# Autodesk Inventor assembly: ROBOT_1_4
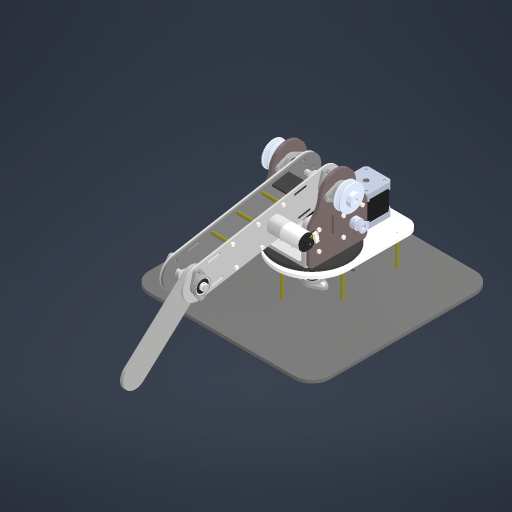
[picture p0: Inventor's stored thumbnail of the model, 512x512]
Saved by Autodesk Inventor 2023 (Build 270158000, 158)
## iProperties
Created: 2023-09-06
Part Number: ROBOT_1_4
Document SubType Name: Assembly
Designer: philo
Sending System: Autodesk Inventor 2023
Preprocessor: ST-DEVELOPER v19
Title: C:\Users\philo\OneDrive\Desktop\HK1-2024\TT ROBOT\3DVer2\ROBOT_1_2.stp
Author: philo
## Documents named in this file (28)
- C:\Users\philo\OneDrive\Desktop\HK1-2024\TT ROBOT\02_3D_design\ROBOT_1_4.iam
- C:\Users\philo\OneDrive\Desktop\HK1-2024\TT ROBOT\02_3D_design\DeRobot.ipt
- C:\Users\philo\OneDrive\Desktop\HK1-2024\TT ROBOT\02_3D_design\Detron.ipt
- C:\Users\philo\OneDrive\Desktop\HK1-2024\TT ROBOT\02_3D_design\goidoObi.ipt
- C:\Users\philo\OneDrive\Desktop\HK1-2024\TT ROBOT\02_3D_design\truday.ipt
- C:\Users\philo\OneDrive\Desktop\HK1-2024\TT ROBOT\02_3D_design\gt2_60teeth.iam
- C:\Users\philo\OneDrive\Desktop\HK1-2024\TT ROBOT\02_3D_design\STEP MOTOR NEMA 17.ipt
- C:\Users\philo\OneDrive\Desktop\HK1-2024\TT ROBOT\02_3D_design\GT2 Pulley 20 Tooth (ID6mm).ipt
- C:\Users\philo\OneDrive\Desktop\HK1-2024\TT ROBOT\02_3D_design\M3 x 5mm.ipt
- C:\Users\philo\OneDrive\Desktop\HK1-2024\TT ROBOT\02_3D_design\Diaquay.ipt
- C:\Users\philo\OneDrive\Desktop\HK1-2024\TT ROBOT\02_3D_design\Tb6600.ipt
- C:\Users\philo\OneDrive\Desktop\HK1-2024\TT ROBOT\02_3D_design\ESP-WROOM32.iam
- C:\Users\philo\OneDrive\Desktop\HK1-2024\TT ROBOT\02_3D_design\codinhtruc.ipt
- C:\Users\philo\OneDrive\Desktop\HK1-2024\TT ROBOT\02_3D_design\daydai.ipt
- C:\Users\philo\OneDrive\Desktop\HK1-2024\TT ROBOT\02_3D_design\gt2smooth.ipt
- C:\Users\philo\OneDrive\Desktop\HK1-2024\TT ROBOT\02_3D_design\trudong5mm.ipt
- C:\Users\philo\OneDrive\Desktop\HK1-2024\TT ROBOT\02_3D_design\trucdogt2.ipt
- C:\Users\philo\OneDrive\Desktop\HK1-2024\TT ROBOT\02_3D_design\HALL.ipt
- C:\Users\philo\OneDrive\Desktop\HK1-2024\TT ROBOT\02_3D_design\namcham.ipt
- C:\Users\philo\OneDrive\Desktop\HK1-2024\TT ROBOT\02_3D_design\Tamop1.ipt
- C:\Users\philo\OneDrive\Desktop\HK1-2024\TT ROBOT\02_3D_design\60pitch pulley GT2 6mm ASSEMBLY.iam
- C:\Users\philo\OneDrive\Desktop\HK1-2024\TT ROBOT\02_3D_design\truc8mm.ipt
- C:\Users\philo\OneDrive\Desktop\HK1-2024\TT ROBOT\02_3D_design\giulink2.ipt
- C:\Users\philo\OneDrive\Desktop\HK1-2024\TT ROBOT\02_3D_design\Link2Base.ipt
- C:\Users\philo\OneDrive\Desktop\HK1-2024\TT ROBOT\02_3D_design\thanhnang.ipt
- C:\Users\philo\OneDrive\Desktop\HK1-2024\TT ROBOT\02_3D_design\trudong3mm.ipt
- C:\Users\philo\OneDrive\Desktop\HK1-2024\TT ROBOT\02_3D_design\Link3base.ipt
- C:\Users\philo\OneDrive\Desktop\HK1-2024\TT ROBOT\02_3D_design\Dongco.iam
## Components (85 placed, 27 different names)
1. Link3base:1 — Mate:171, Flush:17
2. Dongco:1 [sub-assembly] — Mate:172, Angle:18
3. DeRobot:1 — Mate:81, Mate:82, Mate:83, Mate:84, Mate:85, Mate:86, Mate:87, Mate:90, Mate:91, Mate:92, Mate:95, ROBOTQUAY, Flush:16
4. Detron:1 — Mate:33, Mate:81, Mate:94, Mate:95, Mate:96, Mate:97, Angle:11
5. goidoObi:1 — Mate:93, Mate:94
6. goidoObi:2 — Mate:89, Mate:92
7. truday:1 — Mate:32, Mate:87, Mate:88, Mate:93, Flush:16
8. gt2_60teeth:1 [sub-assembly] — Mate:88, Mate:89
9. STEP MOTOR NEMA 17:1 — Mate:96, Mate:97, Angle:11, Mate:98
10. GT2 Pulley 20 Tooth (ID6mm):1 — Mate:98
11. M3 x 5mm:1
12. M3 x 5mm:6
13. M3 x 5mm:7 — Mate:90
14. M3 x 5mm:8 — Mate:91
15. Tb6600:1
16. Tb6600:2
17. ESP-WROOM32:1 [sub-assembly]
18. daydai:1
19. gt2smooth:1 — Mate:99
20. trudong5mm:4 — Mate:84
21. trudong5mm:5 — Mate:82
22. trudong5mm:6 — Mate:85
23. trudong5mm:8 — Mate:86
24. trudong5mm:9 — Mate:83
25. trucdogt2:1 — Mate:99
26. HALL:1
27. goidoObi:5 — Mate:100, Mate:101
28. M3 x 5mm:9 — Mate:38, Mate:56
29. M3 x 5mm:10 — Mate:39, Mate:58
30. M3 x 5mm:11 — Mate:37, Mate:60
31. M3 x 5mm:12 — Mate:40, Mate:57
32. M3 x 5mm:13 — Mate:41, Mate:61
33. M3 x 5mm:14 — Mate:42, Mate:59
34. M3 x 5mm:15 — Mate:43, Mate:52
35. M3 x 5mm:16 — Mate:45, Mate:51
36. M3 x 5mm:17 — Mate:46, Mate:54
37. M3 x 5mm:18 — Mate:44, Mate:50
38. M3 x 5mm:19 — Mate:47, Mate:53
39. M3 x 5mm:20 — Mate:48, Mate:55
40. gt2smooth:2 — Mate:49
41. giulink2:1 — Mate:63, Angle:4, Angle:5, Angle:6, Angle:8, Mate:64, Mate:65, Mate:67, Flush:4, Flush:5, Mate:68, Mate:69, Angle:13, ROBOTQUAY
42. Diaquay:1 — Mate:1, Mate:2, Mate:7, Mate:8, Mate:32, Mate:33, Mate:34, Flush:3, Angle:13, Mate:116, Mate:117
43. codinhtruc:2 — Mate:1, Mate:2, Mate:34, Mate:63
44. namcham:1 — Flush:3, Mate:116, Mate:117
45. STEP MOTOR NEMA 17:2 — Mate:27, Mate:28, Angle:6, Mate:66, Mate:67
46. STEP MOTOR NEMA 17:3 — Mate:26, Mate:30, Angle:5, Angle:8, Mate:64, Mate:65
47. Tamop1:1 — Mate:7, Flush:1, Mate:27, Mate:29, Mate:37, Mate:38, Mate:39, Mate:40, Mate:41, Mate:42, Mate:56, Mate:57, Mate:58, Mate:59, Mate:60, Mate:61, Mate:66, Flush:4, Mate:69, Mate:100, Mate:103, Mate:105, Mate:127
48. GT2 Pulley 20 Tooth (ID6mm):2 — Mate:28, Mate:29
49. 60pitch pulley GT2 6mm ASSEMBLY:1 [sub-assembly] — Mate:102, Mate:103
50. Tamop1:2 — Mate:8, Mate:12, Mate:13, Mate:16, Mate:19, Mate:26, Mate:31, Mate:43, Mate:44, Mate:45, Mate:46, Mate:47, Mate:48, Mate:49, Mate:50, Mate:51, Mate:52, Mate:53, Mate:54, Mate:55, Angle:4, Flush:5, Mate:68, LINK1ANGLE
51. goidoObi:4 — Mate:12, Mate:13, Mate:16, Mate:17
52. GT2 Pulley 20 Tooth (ID6mm):3 — Mate:30, Mate:31
53. 60pitch pulley GT2 6mm ASSEMBLY:2 [sub-assembly] — Mate:19, Mate:20
54. truc8mm:1 — Mate:23, Flush:1, Mate:73, Flush:8, Mate:101, Mate:102, Mate:104, Mate:105, Mate:106
55. truc8mm:2 — Mate:17, Mate:20, Mate:23, Mate:70, Mate:74, Mate:169
56. trudong3mm:1 — Mate:131, Mate:132
57. trudong3mm:3 — Mate:136, Mate:139
58. trudong3mm:4 — Mate:133, Mate:141
59. trudong3mm:5 — Mate:134, Mate:140
60. trudong3mm:6 — Mate:137, Mate:138
61. trudong3mm:7 — Mate:142, Mate:143
62. M3 x 5mm:21 — Mate:144, Mate:145
63. M3 x 5mm:22 — Mate:146, Mate:152
64. M3 x 5mm:23 — Mate:147, Mate:151
65. M3 x 5mm:24 — Mate:148, Mate:150
66. M3 x 5mm:25 — Mate:149, Mate:153
67. M3 x 5mm:26 — Mate:154, Mate:155
68. M3 x 5mm:27 — Mate:156, Mate:159
69. M3 x 5mm:28 — Mate:157, Mate:158
70. M3 x 5mm:29 — Mate:162, Mate:166
71. M3 x 5mm:30 — Mate:160, Mate:167
72. M3 x 5mm:31 — Mate:161, Mate:165
73. M3 x 5mm:32 — Mate:163, Mate:164
74. codinhtruc:4 — Mate:168, Mate:169, Angle:17
75. goidoObi:7 — Mate:118, Mate:119, Angle:15, Flush:15
76. goidoObi:8 — Mate:120, Mate:121, Angle:16, Mate:126
77. truc8mm:3 — Mate:126, Flush:15, Mate:130, Mate:171
78. GT2 Pulley 20 Tooth (ID6mm):5 — Mate:130, Mate:170
79. Link2Base:3 — Mate:106, Mate:107, Mate:108, Mate:109, Mate:110, Flush:12, Mate:118, Mate:119, Angle:15, Angle:16, Mate:122, Mate:127, Mate:132, Mate:133, Mate:134, Mate:136, Mate:137, Mate:138, Mate:139, Mate:140, Mate:141, Mate:144, Mate:145, Mate:146, Mate:147, Mate:148, Mate:149, Mate:150, Mate:151, Mate:152, Mate:153, Mate:154, Mate:155, Angle:17, Mate:170, Flush:17, Mate:172, Angle:18
80. thanhnang:1 — Flush:10, Flush:11, Mate:109
81. thanhnang:2 — Mate:110, Flush:12, Mate:111
82. goidoObi:6 — Mate:104, Mate:107, Mate:122
83. GT2 Pulley 20 Tooth (ID6mm):4 — Mate:73, Flush:8
84. Link2Base:2 — Mate:74, Mate:75, Mate:76, Mate:108, Flush:10, Flush:11, Mate:131, Mate:143
85. Link2Base:1 — Mate:70, LINK1ANGLE, Mate:75, Mate:76, Mate:111, Mate:120, Mate:121, Mate:142, Mate:156, Mate:157, Mate:158, Mate:159, Mate:160, Mate:161, Mate:162, Mate:163, Mate:164, Mate:165, Mate:166, Mate:167, Mate:168
## Relationships (162: Mate 139, Angle 12, Flush 11)
- Mate:1: Diaquay:1 ↔ codinhtruc:2
- Mate:2: Diaquay:1 ↔ codinhtruc:2
- Mate:7: Diaquay:1 ↔ Tamop1:1
- Mate:8: Diaquay:1 ↔ Tamop1:2
- Mate:12: Tamop1:2 ↔ goidoObi:4
- Mate:13: Tamop1:2 ↔ goidoObi:4
- Mate:16: Tamop1:2 ↔ goidoObi:4
- Mate:17: goidoObi:4 ↔ truc8mm:2
- Mate:19 (3 mm): Tamop1:2 ↔ 60pitch pulley GT2 6mm ASSEMBLY:2
- Mate:20: 60pitch pulley GT2 6mm ASSEMBLY:2 ↔ truc8mm:2
- Mate:23 (5 mm): truc8mm:1 ↔ truc8mm:2
- Flush:1 (-36 mm): Tamop1:1 ↔ truc8mm:1
- Mate:26: STEP MOTOR NEMA 17:3 ↔ Tamop1:2
- Mate:27: STEP MOTOR NEMA 17:2 ↔ Tamop1:1
- Mate:28: STEP MOTOR NEMA 17:2 ↔ GT2 Pulley 20 Tooth (ID6mm):2
- Mate:29 (3 mm): Tamop1:1 ↔ GT2 Pulley 20 Tooth (ID6mm):2
- Mate:30: STEP MOTOR NEMA 17:3 ↔ GT2 Pulley 20 Tooth (ID6mm):3
- Mate:31 (3 mm): Tamop1:2 ↔ GT2 Pulley 20 Tooth (ID6mm):3
- Mate:32: truday:1 ↔ Diaquay:1
- Mate:33 (6 mm): Detron:1 ↔ Diaquay:1
- Mate:34: Diaquay:1 ↔ codinhtruc:2
- Mate:37: M3 x 5mm:11 ↔ Tamop1:1
- Mate:38: M3 x 5mm:9 ↔ Tamop1:1
- Mate:39: M3 x 5mm:10 ↔ Tamop1:1
- Mate:40: M3 x 5mm:12 ↔ Tamop1:1
- Mate:41: M3 x 5mm:13 ↔ Tamop1:1
- Mate:42: M3 x 5mm:14 ↔ Tamop1:1
- Mate:43: M3 x 5mm:15 ↔ Tamop1:2
- Mate:44: M3 x 5mm:18 ↔ Tamop1:2
- Mate:45: M3 x 5mm:16 ↔ Tamop1:2
- Mate:46: M3 x 5mm:17 ↔ Tamop1:2
- Mate:47: M3 x 5mm:19 ↔ Tamop1:2
- Mate:48: M3 x 5mm:20 ↔ Tamop1:2
- Mate:49 (8 mm): gt2smooth:2 ↔ Tamop1:2
- Mate:50: M3 x 5mm:18 ↔ Tamop1:2
- Mate:51: M3 x 5mm:16 ↔ Tamop1:2
- Mate:52: M3 x 5mm:15 ↔ Tamop1:2
- Mate:53: M3 x 5mm:19 ↔ Tamop1:2
- Mate:54: M3 x 5mm:17 ↔ Tamop1:2
- Mate:55: M3 x 5mm:20 ↔ Tamop1:2
- Mate:56: M3 x 5mm:9 ↔ Tamop1:1
- Mate:57: M3 x 5mm:12 ↔ Tamop1:1
- Mate:58: M3 x 5mm:10 ↔ Tamop1:1
- Mate:59: M3 x 5mm:14 ↔ Tamop1:1
- Mate:60: M3 x 5mm:11 ↔ Tamop1:1
- Mate:61: M3 x 5mm:13 ↔ Tamop1:1
- Flush:3: Diaquay:1 ↔ namcham:1
- Mate:63: giulink2:1 ↔ codinhtruc:2
- Angle:4 (90 deg): giulink2:1 ↔ Tamop1:2
- Angle:5 (0 deg): giulink2:1 ↔ STEP MOTOR NEMA 17:3
- Angle:6 (0 deg): giulink2:1 ↔ STEP MOTOR NEMA 17:2
- Angle:8 (0 deg): giulink2:1 ↔ STEP MOTOR NEMA 17:3
- Mate:64: giulink2:1 ↔ STEP MOTOR NEMA 17:3
- Mate:65: giulink2:1 ↔ STEP MOTOR NEMA 17:3
- Mate:66: STEP MOTOR NEMA 17:2 ↔ Tamop1:1
- Mate:67: giulink2:1 ↔ STEP MOTOR NEMA 17:2
- Flush:4: giulink2:1 ↔ Tamop1:1
- Flush:5: giulink2:1 ↔ Tamop1:2
- Mate:68: giulink2:1 ↔ Tamop1:2
- Mate:69: giulink2:1 ↔ Tamop1:1
- Mate:70: truc8mm:2 ↔ Link2Base:1
- Mate:73: truc8mm:1 ↔ GT2 Pulley 20 Tooth (ID6mm):4
- Flush:8: truc8mm:1 ↔ GT2 Pulley 20 Tooth (ID6mm):4
- LINK1ANGLE [Angle] (-100 deg): Tamop1:2 ↔ Link2Base:1
- Mate:74: truc8mm:2 ↔ Link2Base:2
- Mate:75: Link2Base:2 ↔ Link2Base:1
- Mate:76: Link2Base:2 ↔ Link2Base:1
- Mate:81 (45 mm): DeRobot:1 ↔ Detron:1
- Mate:82: DeRobot:1 ↔ trudong5mm:5
- Mate:83: DeRobot:1 ↔ trudong5mm:9
- Mate:84: DeRobot:1 ↔ trudong5mm:4
- Mate:85: DeRobot:1 ↔ trudong5mm:6
- Mate:86: DeRobot:1 ↔ trudong5mm:8
- Mate:87: DeRobot:1 ↔ truday:1
- Mate:88: truday:1 ↔ gt2_60teeth:1
- Mate:89: goidoObi:2 ↔ gt2_60teeth:1
- Mate:90: DeRobot:1 ↔ M3 x 5mm:7
- Mate:91: DeRobot:1 ↔ M3 x 5mm:8
- Mate:92: DeRobot:1 ↔ goidoObi:2
- Mate:93: goidoObi:1 ↔ truday:1
- Mate:94: Detron:1 ↔ goidoObi:1
- Mate:95: DeRobot:1 ↔ Detron:1
- Mate:96: Detron:1 ↔ STEP MOTOR NEMA 17:1
- Mate:97: Detron:1 ↔ STEP MOTOR NEMA 17:1
- Angle:11 (0 deg): Detron:1 ↔ STEP MOTOR NEMA 17:1
- Mate:98: STEP MOTOR NEMA 17:1 ↔ GT2 Pulley 20 Tooth (ID6mm):1
- Mate:99: gt2smooth:1 ↔ trucdogt2:1
- Mate:100: goidoObi:5 ↔ Tamop1:1
- Mate:101: goidoObi:5 ↔ truc8mm:1
- Mate:102: 60pitch pulley GT2 6mm ASSEMBLY:1 ↔ truc8mm:1
- Mate:103 (12 mm): Tamop1:1 ↔ 60pitch pulley GT2 6mm ASSEMBLY:1
- Mate:104: truc8mm:1 ↔ goidoObi:6
- Mate:105: Tamop1:1 ↔ truc8mm:1
- Angle:13 (90 deg): giulink2:1 ↔ Diaquay:1
- ROBOTQUAY [Angle] (0 deg): DeRobot:1 ↔ giulink2:1
- Mate:106: truc8mm:1 ↔ Link2Base:3
- Mate:107: Link2Base:3 ↔ goidoObi:6
- Mate:108 (30 mm): Link2Base:3 ↔ Link2Base:2
- Flush:10: thanhnang:1 ↔ Link2Base:2
- Flush:11: thanhnang:1 ↔ Link2Base:2
- Mate:109: Link2Base:3 ↔ thanhnang:1
- Mate:110: Link2Base:3 ↔ thanhnang:2
- Flush:12: Link2Base:3 ↔ thanhnang:2
- Mate:111: thanhnang:2 ↔ Link2Base:1
- Mate:116: Diaquay:1 ↔ namcham:1
- Mate:117 (60 mm): Diaquay:1 ↔ namcham:1
- Mate:118: goidoObi:7 ↔ Link2Base:3
- Mate:119: goidoObi:7 ↔ Link2Base:3
- Angle:15 (90 deg): goidoObi:7 ↔ Link2Base:3
- Mate:120: goidoObi:8 ↔ Link2Base:1
- Mate:121: goidoObi:8 ↔ Link2Base:1
- Angle:16 (90 deg): goidoObi:8 ↔ Link2Base:3
- Mate:122: Link2Base:3 ↔ goidoObi:6
- Mate:126: goidoObi:8 ↔ truc8mm:3
- Flush:15 (-2 mm): goidoObi:7 ↔ truc8mm:3
- Mate:127 (15 mm): Tamop1:1 ↔ Link2Base:3
- Mate:130: truc8mm:3 ↔ GT2 Pulley 20 Tooth (ID6mm):5
- Flush:16: DeRobot:1 ↔ truday:1
- Mate:131: trudong3mm:1 ↔ Link2Base:2
- Mate:132: trudong3mm:1 ↔ Link2Base:3
- Mate:133: trudong3mm:4 ↔ Link2Base:3
- Mate:134: trudong3mm:5 ↔ Link2Base:3
- Mate:136: trudong3mm:3 ↔ Link2Base:3
- Mate:137: trudong3mm:6 ↔ Link2Base:3
- Mate:138: trudong3mm:6 ↔ Link2Base:3
- Mate:139: trudong3mm:3 ↔ Link2Base:3
- Mate:140: trudong3mm:5 ↔ Link2Base:3
- Mate:141: trudong3mm:4 ↔ Link2Base:3
- Mate:142: trudong3mm:7 ↔ Link2Base:1
- Mate:143: trudong3mm:7 ↔ Link2Base:2
- Mate:144: M3 x 5mm:21 ↔ Link2Base:3
- Mate:145: M3 x 5mm:21 ↔ Link2Base:3
- Mate:146: M3 x 5mm:22 ↔ Link2Base:3
- Mate:147: M3 x 5mm:23 ↔ Link2Base:3
- Mate:148: M3 x 5mm:24 ↔ Link2Base:3
- Mate:149: M3 x 5mm:25 ↔ Link2Base:3
- Mate:150: M3 x 5mm:24 ↔ Link2Base:3
- Mate:151: M3 x 5mm:23 ↔ Link2Base:3
- Mate:152: M3 x 5mm:22 ↔ Link2Base:3
- Mate:153: M3 x 5mm:25 ↔ Link2Base:3
- Mate:154: M3 x 5mm:26 ↔ Link2Base:3
- Mate:155: M3 x 5mm:26 ↔ Link2Base:3
- Mate:156: M3 x 5mm:27 ↔ Link2Base:1
- Mate:157: M3 x 5mm:28 ↔ Link2Base:1
- Mate:158: M3 x 5mm:28 ↔ Link2Base:1
- Mate:159: M3 x 5mm:27 ↔ Link2Base:1
- Mate:160: M3 x 5mm:30 ↔ Link2Base:1
- Mate:161: M3 x 5mm:31 ↔ Link2Base:1
- Mate:162: M3 x 5mm:29 ↔ Link2Base:1
- Mate:163: M3 x 5mm:32 ↔ Link2Base:1
- Mate:164: M3 x 5mm:32 ↔ Link2Base:1
- Mate:165: M3 x 5mm:31 ↔ Link2Base:1
- Mate:166: M3 x 5mm:29 ↔ Link2Base:1
- Mate:167: M3 x 5mm:30 ↔ Link2Base:1
- Mate:168: codinhtruc:4 ↔ Link2Base:1
- Mate:169: truc8mm:2 ↔ codinhtruc:4
- Angle:17 (0 deg): codinhtruc:4 ↔ Link2Base:3
- Mate:170 (5 mm): GT2 Pulley 20 Tooth (ID6mm):5 ↔ Link2Base:3
- Mate:171: Link3base:1 ↔ truc8mm:3
- Flush:17 (-10 mm): Link3base:1 ↔ Link2Base:3
- Mate:172: Dongco:1 ↔ Link2Base:3
- Angle:18 (0 deg): Dongco:1 ↔ Link2Base:3
